# Autodesk Inventor assembly: WobbleGripper
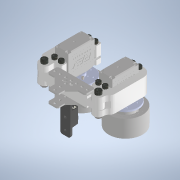
[picture p0: Inventor's stored thumbnail of the model, 180x180]
Saved by Autodesk Inventor 2021 (Build 250183000, 183)
## iProperties
Created: 2021-05-26
Part Number: WobbleGripper
Document SubType Name: Assembly
Designer: sami8
Author: sami8
## Documents named in this file (14)
- C:\Users\sami8\Documents\SGD-FTC2021\CAD\WobbleGripper.iam
- C:\Users\sami8\Documents\FTC 2021\CAD\Intake\REV-41-1097.ipt
- C:\Users\sami8\Documents\FTC 2021\CAD\Intake\REV-41-1125.ipt
- C:\Users\sami8\Documents\FTC 2021\CAD\Intake\REV-41-1846.ipt
- C:\Users\sami8\Documents\FTC 2021\CAD\Intake\am-3664 2in 5mm Hex Bore Stealth Wheel REV3.ipt
- C:\Users\sami8\Documents\SGD-FTC2021\CAD\FloorRoller\REV-41-1363.ipt
- C:\Users\sami8\Documents\SGD-FTC2021\CAD\ServoArm.ipt
- C:\Users\sami8\Documents\SGD-FTC2021\CAD\ServoArm_MIR.ipt
- C:\Users\sami8\Documents\SGD-FTC2021\CAD\WobbleGripper\M4x0.7_25mm_91290A176.ipt
- C:\Users\sami8\Documents\SGD-FTC2021\CAD\RearArm.ipt
- C:\Users\sami8\Documents\SGD-FTC2021\CAD\WobbleGripper\M5x0.8_30mm_91290A254.ipt
- C:\Users\sami8\Documents\SGD-FTC2021\CAD\WobbleGripper\M5x0.8mm_NYLOCK_90576A104.ipt
- C:\Users\sami8\Documents\SGD-FTC2021\CAD\WobbleGripper\REV-41-1483.ipt
- C:\Users\sami8\Documents\SGD-FTC2021\CAD\WobbleGripper\REV-31-1425.ipt
## Components (32 placed, 13 different names)
1. REV-41-1097:1 — Rigid:1, Mate:1, Mate:2, Mate:3, Angle:1
2. REV-41-1125:1 — Rigid:5
3. REV-41-1846:1 — Rigid:2, Rigid:3
4. am-3664 2in 5mm Hex Bore Stealth Wheel REV3:1 — Rigid:4, Rigid:5, Rigid:6
5. REV-41-1363:1 — Rigid:1, Rigid:2
6. REV-41-1846:2 — Rigid:3, Rigid:4
7. REV-41-1125:2 — Rigid:6
8. ServoArm:1 — Mate:1, Mate:2, Mate:3, Rigid:7, Rigid:8, Rigid:9, Rigid:10, Angle:1, Rotational:1, Rigid:21, Rigid:22
9. ServoArm_MIR:1 — Mate:4, Mate:5, Mate:6, Rigid:17, Rigid:18, Rigid:19, Rigid:20, Angle:2, Rotational:2, Rigid:23, Rigid:24
10. M4x0.7_25mm_91290A176:1 — Rigid:7
11. M4x0.7_25mm_91290A176:2 — Rigid:8
12. M4x0.7_25mm_91290A176:3 — Rigid:9
13. M4x0.7_25mm_91290A176:4 — Rigid:10
14. REV-41-1097:2 — Mate:4, Mate:5, Mate:6, Angle:2
15. REV-41-1125:3
16. REV-41-1846:3
17. am-3664 2in 5mm Hex Bore Stealth Wheel REV3:2
18. REV-41-1363:2
19. REV-41-1846:4
20. REV-41-1125:4
21. M4x0.7_25mm_91290A176:5 — Rigid:17
22. M4x0.7_25mm_91290A176:6 — Rigid:18
23. M4x0.7_25mm_91290A176:7 — Rigid:20
24. M4x0.7_25mm_91290A176:8 — Rigid:19
25. RearArm:1 — Rotational:1, Rotational:2, Rigid:25, Rigid:26
26. M5x0.8_30mm_91290A254:1 — Rigid:21
27. M5x0.8mm_NYLOCK_90576A104:1 — Rigid:22
28. M5x0.8_30mm_91290A254:2 — Rigid:23
29. M5x0.8mm_NYLOCK_90576A104:2 — Rigid:24
30. REV-41-1483:1 — Rigid:25
31. REV-41-1483:2 — Rigid:26
32. REV-31-1425:1
## Relationships (36: WeldJoint 26, Mate 6, Angle 2, RevoluteJoint 2)
- Rigid:1 [WeldJoint]: REV-41-1097:1 ↔ REV-41-1363:1
- Rigid:2 [WeldJoint]: REV-41-1846:1 ↔ REV-41-1363:1
- Rigid:3 [WeldJoint]: REV-41-1846:1 ↔ REV-41-1846:2
- Rigid:4 [WeldJoint]: am-3664 2in 5mm Hex Bore Stealth Wheel REV3:1 ↔ REV-41-1846:2
- Rigid:5 [WeldJoint]: REV-41-1125:1 ↔ am-3664 2in 5mm Hex Bore Stealth Wheel REV3:1
- Rigid:6 [WeldJoint]: am-3664 2in 5mm Hex Bore Stealth Wheel REV3:1 ↔ REV-41-1125:2
- Mate:1: REV-41-1097:1 ↔ ServoArm:1
- Mate:2 (-3 mm): REV-41-1097:1 ↔ ServoArm:1
- Mate:3: REV-41-1097:1 ↔ ServoArm:1
- Rigid:7 [WeldJoint]: ServoArm:1 ↔ M4x0.7_25mm_91290A176:1
- Rigid:8 [WeldJoint]: ServoArm:1 ↔ M4x0.7_25mm_91290A176:2
- Rigid:9 [WeldJoint]: ServoArm:1 ↔ M4x0.7_25mm_91290A176:3
- Rigid:10 [WeldJoint]: ServoArm:1 ↔ M4x0.7_25mm_91290A176:4
- [WeldJoint]: REV-41-1097:2 ↔ REV-41-1363:2
- [WeldJoint]: REV-41-1846:3 ↔ REV-41-1363:2
- [WeldJoint]: REV-41-1846:3 ↔ REV-41-1846:4
- [WeldJoint]: am-3664 2in 5mm Hex Bore Stealth Wheel REV3:2 ↔ REV-41-1846:4
- [WeldJoint]: REV-41-1125:3 ↔ am-3664 2in 5mm Hex Bore Stealth Wheel REV3:2
- [WeldJoint]: am-3664 2in 5mm Hex Bore Stealth Wheel REV3:2 ↔ REV-41-1125:4
- Mate:4: ServoArm_MIR:1 ↔ REV-41-1097:2
- Mate:5 (-3 mm): ServoArm_MIR:1 ↔ REV-41-1097:2
- Mate:6: ServoArm_MIR:1 ↔ REV-41-1097:2
- Rigid:17 [WeldJoint]: ServoArm_MIR:1 ↔ M4x0.7_25mm_91290A176:5
- Rigid:18 [WeldJoint]: ServoArm_MIR:1 ↔ M4x0.7_25mm_91290A176:6
- Rigid:19 [WeldJoint]: ServoArm_MIR:1 ↔ M4x0.7_25mm_91290A176:8
- Rigid:20 [WeldJoint]: ServoArm_MIR:1 ↔ M4x0.7_25mm_91290A176:7
- Angle:1 (180.5 deg): REV-41-1097:1 ↔ ServoArm:1
- Angle:2 (180.5 deg): ServoArm_MIR:1 ↔ REV-41-1097:2
- Rotational:1 [RevoluteJoint] (-0.25 mm): ServoArm:1 ↔ RearArm:1
- Rotational:2 [RevoluteJoint] (-0.25 mm): ServoArm_MIR:1 ↔ RearArm:1
- Rigid:21 [WeldJoint]: ServoArm:1 ↔ M5x0.8_30mm_91290A254:1
- Rigid:22 [WeldJoint]: ServoArm:1 ↔ M5x0.8mm_NYLOCK_90576A104:1
- Rigid:23 [WeldJoint]: ServoArm_MIR:1 ↔ M5x0.8_30mm_91290A254:2
- Rigid:24 [WeldJoint]: ServoArm_MIR:1 ↔ M5x0.8mm_NYLOCK_90576A104:2
- Rigid:25 [WeldJoint]: RearArm:1 ↔ REV-41-1483:1
- Rigid:26 [WeldJoint]: RearArm:1 ↔ REV-41-1483:2
## Named parameters: d15_d3 = 0 mm, d16_d4 = 0 mm, d17_d5 = 0 mm, d18_d0 = 0 mm, d19_d1 = 0 mm, d20_d2 = 0 mm
